# Autodesk Inventor assembly: torsosc-container-4drawing
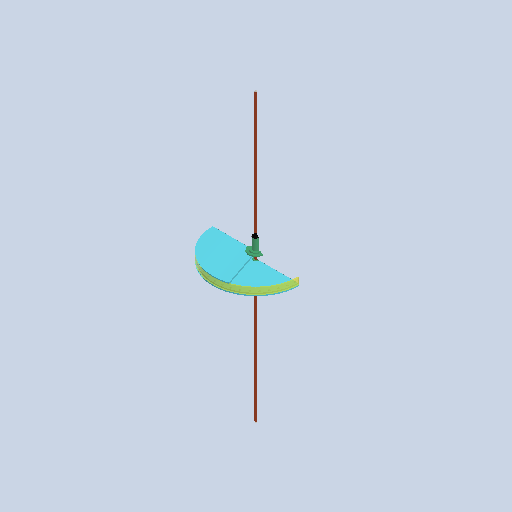
[picture p0: Inventor's stored thumbnail of the model, 512x512]
Saved by Autodesk Inventor 2026 (Build 300175050, 175E)
## iProperties
Created: 2025-11-28
Part Number: torsosc-container-4drawing
Document SubType Name: Assembly
Designer: schanen
Author: schanen
## Documents named in this file (9)
- C:\Users\schanen\Documents\work-experiments-torsosc-2026\inventor\torsosc-container-4drawing.iam
- C:\Users\schanen\Documents\work-experiments-torsosc-2026\inventor\torsosc-container-wall.ipt
- C:\Users\schanen\Documents\work-experiments-torsosc-2026\inventor\torsosc-container-plate.ipt
- C:\Users\schanen\Documents\work-experiments-torsosc-2026\inventor\torsosc-container-tower.ipt
- C:\Users\schanen\Documents\work-experiments-torsosc-2026\inventor\torsosc-torsionrod.ipt
- C:\Users\schanen\Documents\work-experiments-torsosc-2026\inventor\torsosc-container-glue-2-torsionrod.ipt
- C:\Users\schanen\Documents\work-experiments-torsosc-2026\inventor\torsosc-container-glue-2-pcb.ipt
- C:\Users\schanen\Documents\work-experiments-torsosc-2026\inventor\torsosc-fillingline-coupling-solder-2-torsionrod.ipt
- C:\Users\schanen\Documents\work-experiments-torsosc-2026\inventor\torsosc-container-plate-4drawing.ipt
## Components (12 placed, 8 different names)
1. torsosc-container-wall:1 — Mate:5, Mate:6, Mate:7, Mate:8, Mate:9
2. torsosc-container-plate:1 — Mate:4, Mate:7, Mate:8, Mate:12, Mate:33, Mate:39
3. torsosc-container-tower:1 — Mate:4, Mate:15, Mate:31, Mate:33, Mate:38
4. torsosc-container-plate-4drawing:1 — Mate:2, Mate:5, Mate:6, Flush:2, Mate:12, Mate:41
5. torsosc-container-tower:2 — Mate:2, Mate:17, Mate:32, Mate:40
6. torsosc-torsionrod:1 — Flush:1, Mate:11, Mate:14, Mate:16, Mate:31, Mate:32, Mate:42, Mate:43, Mate:44, Mate:45
7. torsosc-container-glue-2-torsionrod:1 — Mate:14, Mate:15
8. torsosc-container-glue-2-torsionrod:2 — Mate:16, Mate:17
9. torsosc-container-glue-2-pcb:1 — Mate:40, Mate:41
10. torsosc-container-glue-2-pcb:2 — Mate:38, Mate:39
11. torsosc-fillingline-coupling-solder-2-torsionrod:1 — Mate:42, Mate:43
12. torsosc-fillingline-coupling-solder-2-torsionrod:2 — Mate:44, Mate:45
## Relationships (26: Mate 24, Flush 2)
- Mate:2: torsosc-container-plate-4drawing:1 ↔ torsosc-container-tower:2
- Mate:4: torsosc-container-plate:1 ↔ torsosc-container-tower:1
- Mate:5: torsosc-container-wall:1 ↔ torsosc-container-plate-4drawing:1
- Mate:6: torsosc-container-wall:1 ↔ torsosc-container-plate-4drawing:1
- Mate:7: torsosc-container-wall:1 ↔ torsosc-container-plate:1
- Mate:8: torsosc-container-wall:1 ↔ torsosc-container-plate:1
- Mate:9: torsosc-container-wall:1
- Flush:1 (-66 mm): torsosc-torsionrod:1
- Flush:2 (-2 mm): torsosc-container-plate-4drawing:1
- Mate:11: torsosc-torsionrod:1
- Mate:12: torsosc-container-plate:1 ↔ torsosc-container-plate-4drawing:1
- Mate:14: torsosc-torsionrod:1 ↔ torsosc-container-glue-2-torsionrod:1
- Mate:15: torsosc-container-tower:1 ↔ torsosc-container-glue-2-torsionrod:1
- Mate:16: torsosc-torsionrod:1 ↔ torsosc-container-glue-2-torsionrod:2
- Mate:17: torsosc-container-tower:2 ↔ torsosc-container-glue-2-torsionrod:2
- Mate:31: torsosc-container-tower:1 ↔ torsosc-torsionrod:1
- Mate:32: torsosc-container-tower:2 ↔ torsosc-torsionrod:1
- Mate:33: torsosc-container-plate:1 ↔ torsosc-container-tower:1
- Mate:38: torsosc-container-tower:1 ↔ torsosc-container-glue-2-pcb:2
- Mate:39: torsosc-container-plate:1 ↔ torsosc-container-glue-2-pcb:2
- Mate:40: torsosc-container-tower:2 ↔ torsosc-container-glue-2-pcb:1
- Mate:41: torsosc-container-plate-4drawing:1 ↔ torsosc-container-glue-2-pcb:1
- Mate:42: torsosc-torsionrod:1 ↔ torsosc-fillingline-coupling-solder-2-torsionrod:1
- Mate:43: torsosc-torsionrod:1 ↔ torsosc-fillingline-coupling-solder-2-torsionrod:1
- Mate:44: torsosc-torsionrod:1 ↔ torsosc-fillingline-coupling-solder-2-torsionrod:2
- Mate:45: torsosc-torsionrod:1 ↔ torsosc-fillingline-coupling-solder-2-torsionrod:2
